# Autodesk Inventor assembly: Stewart-Base-KST-DS215
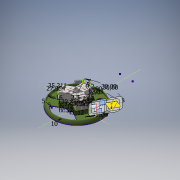
[picture p0: Inventor's stored thumbnail of the model, 180x180]
Saved by Autodesk Inventor 2018.2 (Build 222227000, 227)
## iProperties
Created: 2018-02-24
Part Number: Stewart-Base-KST-DS215
Material: Generisch
Document SubType Name: Assembly
Designer: JochenAlt
Author: JochenAlt
## Documents named in this file (5)
- D:\Projects\Donna\CAD\Stewart-Base.iam
- D:\Projects\Donna\CAD\Stewart-Platform-Base.ipt
- D:\Projects\Donna\CAD\Servo-KST-DS215MG.ipt
- D:\Projects\Donna\CAD\Messung.ipt
- D:\Projects\Donna\CAD\Servo-Arm-Head-20mm-Ball-Joint.iam
## Components (9 placed, 4 different names)
1. Stewart-Platform-Base-KST-DS215MG:1 — Passend:34, Passend:36, Passend:37, Passend:38, Passend:39, Passend:45, Passend:46, Passend:49, Passend:50, Passend:53, Passend:54, Passend:55, Passend:56, Passend:57, Passend:58, Passend:59, Passend:60, Passend:61, Passend:62, Passend:63, Passend:66
2. Servo-KST-DS215MG:1 — Passend:36, Passend:38, Passend:63
3. Servo-KST-DS215MG:2 — Passend:37, Passend:39, Passend:62
4. Servo-KST-DS215MG:3 — Passend:45, Passend:54, Passend:56
5. Servo-KST-DS215MG:4 — Passend:46, Passend:53, Passend:55
6. Servo-KST-DS215MG:5 — Passend:49, Passend:58, Passend:59
7. Servo-KST-DS215MG:6 — Passend:50, Passend:57, Passend:60, Passend:67, Passend:68
8. Servo-Arm-Head-20mm-Ball-Joint:1 [sub-assembly] — Passend:67, Passend:68
9. Messung:1 — Fluchtend:1
## Relationships (24: Mate 23, Flush 1)
- Passend:34 [Mate]: Stewart-Platform-Base-KST-DS215MG:1
- Passend:36 [Mate]: Stewart-Platform-Base-KST-DS215MG:1 ↔ Servo-KST-DS215MG:1
- Passend:37 [Mate]: Stewart-Platform-Base-KST-DS215MG:1 ↔ Servo-KST-DS215MG:2
- Passend:38 [Mate]: Stewart-Platform-Base-KST-DS215MG:1 ↔ Servo-KST-DS215MG:1
- Passend:39 [Mate]: Stewart-Platform-Base-KST-DS215MG:1 ↔ Servo-KST-DS215MG:2
- Passend:45 [Mate]: Stewart-Platform-Base-KST-DS215MG:1 ↔ Servo-KST-DS215MG:3
- Passend:46 [Mate]: Stewart-Platform-Base-KST-DS215MG:1 ↔ Servo-KST-DS215MG:4
- Passend:49 [Mate]: Stewart-Platform-Base-KST-DS215MG:1 ↔ Servo-KST-DS215MG:5
- Passend:50 [Mate]: Stewart-Platform-Base-KST-DS215MG:1 ↔ Servo-KST-DS215MG:6
- Passend:53 [Mate]: Stewart-Platform-Base-KST-DS215MG:1 ↔ Servo-KST-DS215MG:4
- Passend:54 [Mate]: Stewart-Platform-Base-KST-DS215MG:1 ↔ Servo-KST-DS215MG:3
- Passend:55 [Mate]: Stewart-Platform-Base-KST-DS215MG:1 ↔ Servo-KST-DS215MG:4
- Passend:56 [Mate]: Stewart-Platform-Base-KST-DS215MG:1 ↔ Servo-KST-DS215MG:3
- Passend:57 [Mate]: Stewart-Platform-Base-KST-DS215MG:1 ↔ Servo-KST-DS215MG:6
- Passend:58 [Mate]: Stewart-Platform-Base-KST-DS215MG:1 ↔ Servo-KST-DS215MG:5
- Passend:59 [Mate]: Stewart-Platform-Base-KST-DS215MG:1 ↔ Servo-KST-DS215MG:5
- Passend:60 [Mate]: Stewart-Platform-Base-KST-DS215MG:1 ↔ Servo-KST-DS215MG:6
- Fluchtend:1 [Flush]: Messung:1
- Passend:61 [Mate]: Stewart-Platform-Base-KST-DS215MG:1
- Passend:62 [Mate]: Stewart-Platform-Base-KST-DS215MG:1 ↔ Servo-KST-DS215MG:2
- Passend:63 [Mate]: Stewart-Platform-Base-KST-DS215MG:1 ↔ Servo-KST-DS215MG:1
- Passend:66 [Mate]: Stewart-Platform-Base-KST-DS215MG:1
- Passend:67 [Mate]: Servo-KST-DS215MG:6 ↔ Servo-Arm-Head-20mm-Ball-Joint:1
- Passend:68 [Mate]: Servo-KST-DS215MG:6 ↔ Servo-Arm-Head-20mm-Ball-Joint:1
